# Autodesk Inventor assembly: Hoverboard
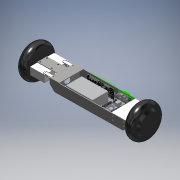
[picture p0: Inventor's stored thumbnail of the model, 180x180]
Saved by Autodesk Inventor 2019.3 (Build 233278000, 278)
## iProperties
Created: 2019-01-26
Part Number: Hoverboard
Document SubType Name: Assembly
Designer: mark
Mass: 13767.9 g
Surface Area: 24732.3 cm^2
Volume: 13767.9 cm^3
Density: 1 g/cm^3
Author: mark
## Documents named in this file (28)
- C:\Users\mark\Documents\Hoverboard\Mechanical\Packed\Hoverboard.iam
- C:\Users\mark\Documents\Hoverboard\Mechanical\Packed\SideBracket.ipt
- C:\Users\mark\Documents\Hoverboard\Mechanical\Packed\LoadCellPlate.ipt
- C:\Users\mark\Documents\Hoverboard\Mechanical\Packed\TorquePlate.ipt
- C:\Users\mark\Documents\Hoverboard\Mechanical\Packed\MotorMountRight.ipt
- C:\Users\mark\Documents\Hoverboard\Mechanical\Packed\MotorMountLeft.ipt
- C:\Users\mark\Documents\Hoverboard\Mechanical\Packed\LoadCell.ipt
- C:\Users\mark\Documents\Hoverboard\Mechanical\Packed\LeftSupportBracket.ipt
- C:\Users\mark\Documents\Hoverboard\Mechanical\Packed\Battery.ipt
- C:\Users\mark\Documents\Hoverboard\Mechanical\Packed\BatteryBracket.ipt
- C:\Users\mark\Documents\Hoverboard\Mechanical\Packed\Wheel.ipt
- C:\Users\mark\Documents\Hoverboard\Mechanical\Packed\BEAGLEBONE_BLACK.STEP.ipt
- C:\Users\mark\Documents\Hoverboard\Mechanical\Packed\MPU 6050 IMU.ipt
- C:\Users\mark\Documents\Hoverboard\Mechanical\Packed\HX711.ipt
- C:\Users\mark\Documents\Hoverboard\Mechanical\Packed\PowerSupply.ipt
- C:\Users\mark\Documents\Hoverboard\Mechanical\Packed\ODrive3.4.ipt
- C:\Users\mark\Documents\Hoverboard\Mechanical\Packed\BatteryBracketLeft.ipt
- C:\Users\mark\Documents\Hoverboard\Mechanical\Packed\HX711MountingBracket.ipt
- C:\Users\mark\Documents\Hoverboard\Mechanical\Packed\motherboard_stand.ipt
- C:\Users\mark\Documents\Hoverboard\Mechanical\OdriveMountingBracket.ipt
- C:\Users\mark\Documents\Hoverboard\Mechanical\PowerMountingBracket.ipt
- C:\Users\mark\Documents\Hoverboard\Mechanical\BeagleBoneMountingBracket.ipt
- C:\Users\mark\Documents\Hoverboard\Mechanical\Packed\crof3oa4g.fins
- C:\Users\mark\Documents\Hoverboard\Mechanical\Packed\crof3oa4g.fsat
- C:\Users\mark\Documents\Hoverboard\Mechanical\Packed\crof3oa68.ftes
- C:\Users\mark\Documents\Hoverboard\Mechanical\Packed\crof3oa68.fwiz
- C:\Users\mark\Documents\Hoverboard\Mechanical\Packed\crof3oa8w.fmsh
- C:\Users\mark\Documents\Hoverboard\Mechanical\Packed\crof3oa8x.fres
## Components (28 placed, 21 different names)
1. MotorMountRight:1 — Mate:1, Mate:2, Mate:3, Mate:4, Flush:4, Insert:8
2. SideBracket:1 — Mate:3, Mate:4, Mate:5, Flush:1, Flush:2, Mate:7, Flush:4, Mate:15, Flush:6
3. SideBracket:2 — Mate:1, Mate:2, Mate:17, Mate:36, Mate:37, Mate:38, Mate:39
4. LoadCellPlate:1 — Mate:5, Flush:1, Flush:2, Mate:6, Mate:8, Mate:9, Mate:10, Mate:11, Mate:14, Flush:5
5. TorquePlate:1 — Mate:6, Mate:7, Mate:16, Mate:17
6. MotorMountLeft:1 — Mate:12, Insert:2, Insert:7, Insert:9
7. LoadCell:1 — Mate:8, Mate:9, Mate:12
8. LoadCell:2 — Mate:10, Mate:11, Insert:7
9. LeftSupportBracket:1 — Mate:14, Flush:5, Insert:2
10. Battery:1 — Insert:3, Insert:4, Insert:5, Insert:6
11. BatteryBracket:1 — Insert:3, Insert:4, Mate:15, Flush:6, Mate:43, Mate:44
12. BatteryBracketLeft:1 — Insert:5, Insert:6, Mate:16, Mate:18, Mate:19, Mate:20
13. Wheel:1 — Insert:8
14. Wheel:2 — Insert:9
15. BEAGLEBONE_BLACK.STEP:1 — Mate:45
16. MPU 6050 IMU:1 — Mate:40
17. HX711:1 — Mate:29, Mate:30
18. HX711:2 — Mate:31, Mate:32
19. PowerSupply:1 — Mate:41, Mate:42
20. ODrive3.4:1 — Mate:33, Mate:34, Mate:35
21. HX711MountingBracket:1 — Mate:18, Mate:19, Mate:20, Mate:21, Mate:22, Mate:23, Mate:24, Mate:25, Mate:26, Mate:27, Mate:28
22. motherboard_stand:1 — Mate:21, Mate:22, Mate:29, Mate:30
23. motherboard_stand:2 — Mate:27, Mate:28
24. motherboard_stand:3 — Mate:23, Mate:24
25. motherboard_stand:4 — Mate:25, Mate:26, Mate:31, Mate:32
26. OdriveMountingBracket:1 — Mate:33, Mate:34, Mate:35, Mate:36, Mate:37
27. PowerMountingBracket:1 — Mate:38, Mate:39, Mate:40, Mate:41, Mate:42
28. BeagleBoneMountingBracket:1 — Mate:43, Mate:44, Mate:45
## Relationships (57: Mate 44, Insert 8, Flush 5)
- Mate:1: MotorMountRight:1 ↔ SideBracket:2
- Mate:2: MotorMountRight:1 ↔ SideBracket:2
- Mate:3: MotorMountRight:1 ↔ SideBracket:1
- Mate:4: MotorMountRight:1 ↔ SideBracket:1
- Mate:5: SideBracket:1 ↔ LoadCellPlate:1
- Flush:1: SideBracket:1 ↔ LoadCellPlate:1
- Flush:2: SideBracket:1 ↔ LoadCellPlate:1
- Mate:6: LoadCellPlate:1 ↔ TorquePlate:1
- Mate:7: SideBracket:1 ↔ TorquePlate:1
- Mate:8: LoadCellPlate:1 ↔ LoadCell:1
- Mate:9: LoadCellPlate:1 ↔ LoadCell:1
- Mate:10: LoadCellPlate:1 ↔ LoadCell:2
- Mate:11: LoadCellPlate:1 ↔ LoadCell:2
- Flush:4: MotorMountRight:1 ↔ SideBracket:1
- Mate:12: MotorMountLeft:1 ↔ LoadCell:1
- Mate:14: LoadCellPlate:1 ↔ LeftSupportBracket:1
- Flush:5: LoadCellPlate:1 ↔ LeftSupportBracket:1
- Insert:2: MotorMountLeft:1 ↔ LeftSupportBracket:1
- Insert:3: Battery:1 ↔ BatteryBracket:1
- Insert:4: Battery:1 ↔ BatteryBracket:1
- Insert:5: Battery:1 ↔ BatteryBracketLeft:1
- Insert:6: Battery:1 ↔ BatteryBracketLeft:1
- Mate:15: SideBracket:1 ↔ BatteryBracket:1
- Flush:6: SideBracket:1 ↔ BatteryBracket:1
- Mate:16: TorquePlate:1 ↔ BatteryBracketLeft:1
- Mate:17: SideBracket:2 ↔ TorquePlate:1
- Insert:7: MotorMountLeft:1 ↔ LoadCell:2
- Insert:8 (-50 mm): MotorMountRight:1 ↔ Wheel:1
- Insert:9 (-50 mm): MotorMountLeft:1 ↔ Wheel:2
- Mate:18: BatteryBracketLeft:1 ↔ HX711MountingBracket:1
- Mate:19: BatteryBracketLeft:1 ↔ HX711MountingBracket:1
- Mate:20: BatteryBracketLeft:1 ↔ HX711MountingBracket:1
- Mate:21: HX711MountingBracket:1 ↔ motherboard_stand:1
- Mate:22: HX711MountingBracket:1 ↔ motherboard_stand:1
- Mate:23: HX711MountingBracket:1 ↔ motherboard_stand:3
- Mate:24: HX711MountingBracket:1 ↔ motherboard_stand:3
- Mate:25: HX711MountingBracket:1 ↔ motherboard_stand:4
- Mate:26: HX711MountingBracket:1 ↔ motherboard_stand:4
- Mate:27: HX711MountingBracket:1 ↔ motherboard_stand:2
- Mate:28: HX711MountingBracket:1 ↔ motherboard_stand:2
- Mate:29: HX711:1 ↔ motherboard_stand:1
- Mate:30: HX711:1 ↔ motherboard_stand:1
- Mate:31: HX711:2 ↔ motherboard_stand:4
- Mate:32: HX711:2 ↔ motherboard_stand:4
- Mate:33: ODrive3.4:1 ↔ OdriveMountingBracket:1
- Mate:34: ODrive3.4:1 ↔ OdriveMountingBracket:1
- Mate:35: ODrive3.4:1 ↔ OdriveMountingBracket:1
- Mate:36: SideBracket:2 ↔ OdriveMountingBracket:1
- Mate:37: SideBracket:2 ↔ OdriveMountingBracket:1
- Mate:38: SideBracket:2 ↔ PowerMountingBracket:1
- Mate:39: SideBracket:2 ↔ PowerMountingBracket:1
- Mate:40: MPU 6050 IMU:1 ↔ PowerMountingBracket:1
- Mate:41: PowerSupply:1 ↔ PowerMountingBracket:1
- Mate:42: PowerSupply:1 ↔ PowerMountingBracket:1
- Mate:43: BatteryBracket:1 ↔ BeagleBoneMountingBracket:1
- Mate:44: BatteryBracket:1 ↔ BeagleBoneMountingBracket:1
- Mate:45: BEAGLEBONE_BLACK.STEP:1 ↔ BeagleBoneMountingBracket:1
## Named parameters: sa_0 = 2.9994e-09, sa_1 = 4788.54, sa_2 = 99885.3, sa_3 = 3.174e-09, sa_4 = 4788.54, sa_5 = 99885.3
note: some values were not read from the file. Shown as the stored number, unit unknown: "sa_0", "sa_1", "sa_2", "sa_3", "sa_4", "sa_5".
